# Autodesk Inventor assembly: FrameAssembly
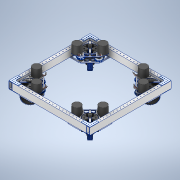
[picture p0: Inventor's stored thumbnail of the model, 180x180]
Saved by Autodesk Inventor 2020 (Build 240168000, 168)
## iProperties
Created: 2019-06-24
Part Number: FrameAssembly
Document SubType Name: Assembly
Designer: Connor
Author: Connor
## Documents named in this file (5)
- C:\Users\Connor\Documents\GrabCAD\2019 Robot\Swerve\TorqyoDriftV2\FrameAssembly.iam
- C:\Users\Connor\Documents\GrabCAD\2019 Robot\Swerve\TorqyoDriftV2\22in2x1Extrusion.ipt
- C:\Users\Connor\Documents\GrabCAD\2019 Robot\Swerve\TorqyoDriftV2\24in2x1Extrusion.ipt
- C:\Users\Connor\Documents\GrabCAD\2019 Robot\Swerve\TorqyoDriftV2\ModuleAssembly.iam
- C:\Users\Connor\Documents\GrabCAD\2019 Robot\Imported Components\VEXPro VersaFrame\General Gussets\90 Degree Gusset.ipt
## Components (16 placed, 4 different names)
1. 22in2x1Extrusion:1 — Mate:1, Flush:1, Flush:2, Flush:6, Flush:11, Flush:13, Insert:2, Insert:9
2. 24in2x1Extrusion:1 — Mate:1, Flush:1, Flush:2, Mate:2, Flush:3, Flush:4, Flush:8, Flush:10, Insert:4, Insert:5, Insert:6, Insert:7, Insert:12, Insert:14, Mate:9, Mate:12, Mate:13
3. 22in2x1Extrusion:2 — Mate:2, Flush:3, Flush:4, Mate:3, Flush:7, Flush:9, Flush:14, Mate:8, Insert:11, Insert:13
4. 24in2x1Extrusion:2 — Flush:6, Mate:3, Flush:7, Flush:12, Flush:15, Insert:1, Insert:3, Insert:8, Insert:10, Mate:10, Mate:11
5. ModuleAssembly:1 [sub-assembly] — Flush:12, Flush:13, Mate:11
6. ModuleAssembly:2 [sub-assembly] — Flush:8, Flush:9, Mate:13
7. ModuleAssembly:3 [sub-assembly] — Flush:14, Flush:15, Mate:10
8. ModuleAssembly:4 [sub-assembly] — Flush:10, Flush:11, Mate:12
9. 90 Degree Gusset:1 — Insert:3, Mate:8
10. 90 Degree Gusset:2 — Insert:8, Insert:9
11. 90 Degree Gusset:3 — Insert:6, Insert:7
12. 90 Degree Gusset:4 — Insert:4, Insert:5
13. 90 Degree Gusset:5 — Insert:10, Insert:11
14. 90 Degree Gusset:6 — Insert:12, Insert:13
15. 90 Degree Gusset:7 — Insert:1, Insert:2
16. 90 Degree Gusset:8 — Insert:14, Mate:9
## Relationships (37: Flush 14, Insert 14, Mate 9)
- Mate:1: 22in2x1Extrusion:1 ↔ 24in2x1Extrusion:1
- Flush:1: 22in2x1Extrusion:1 ↔ 24in2x1Extrusion:1
- Flush:2: 22in2x1Extrusion:1 ↔ 24in2x1Extrusion:1
- Mate:2: 24in2x1Extrusion:1 ↔ 22in2x1Extrusion:2
- Flush:3: 24in2x1Extrusion:1 ↔ 22in2x1Extrusion:2
- Flush:4: 24in2x1Extrusion:1 ↔ 22in2x1Extrusion:2
- Flush:6: 22in2x1Extrusion:1 ↔ 24in2x1Extrusion:2
- Mate:3: 22in2x1Extrusion:2 ↔ 24in2x1Extrusion:2
- Flush:7: 22in2x1Extrusion:2 ↔ 24in2x1Extrusion:2
- Flush:8: 24in2x1Extrusion:1 ↔ ModuleAssembly:2
- Flush:9: 22in2x1Extrusion:2 ↔ ModuleAssembly:2
- Flush:10: 24in2x1Extrusion:1 ↔ ModuleAssembly:4
- Flush:11: 22in2x1Extrusion:1 ↔ ModuleAssembly:4
- Flush:12: 24in2x1Extrusion:2 ↔ ModuleAssembly:1
- Flush:13: 22in2x1Extrusion:1 ↔ ModuleAssembly:1
- Flush:14: 22in2x1Extrusion:2 ↔ ModuleAssembly:3
- Flush:15: 24in2x1Extrusion:2 ↔ ModuleAssembly:3
- Insert:1: 24in2x1Extrusion:2 ↔ 90 Degree Gusset:7
- Insert:2: 22in2x1Extrusion:1 ↔ 90 Degree Gusset:7
- Insert:3: 24in2x1Extrusion:2 ↔ 90 Degree Gusset:1
- Mate:8: 22in2x1Extrusion:2 ↔ 90 Degree Gusset:1
- Insert:4: 24in2x1Extrusion:1 ↔ 90 Degree Gusset:4
- Insert:5: 24in2x1Extrusion:1 ↔ 90 Degree Gusset:4
- Insert:6: 24in2x1Extrusion:1 ↔ 90 Degree Gusset:3
- Insert:7: 24in2x1Extrusion:1 ↔ 90 Degree Gusset:3
- Insert:8: 24in2x1Extrusion:2 ↔ 90 Degree Gusset:2
- Insert:9: 22in2x1Extrusion:1 ↔ 90 Degree Gusset:2
- Insert:10: 24in2x1Extrusion:2 ↔ 90 Degree Gusset:5
- Insert:11: 22in2x1Extrusion:2 ↔ 90 Degree Gusset:5
- Insert:12: 24in2x1Extrusion:1 ↔ 90 Degree Gusset:6
- Insert:13: 22in2x1Extrusion:2 ↔ 90 Degree Gusset:6
- Insert:14: 24in2x1Extrusion:1 ↔ 90 Degree Gusset:8
- Mate:9: 24in2x1Extrusion:1 ↔ 90 Degree Gusset:8
- Mate:10: 24in2x1Extrusion:2 ↔ ModuleAssembly:3
- Mate:11: 24in2x1Extrusion:2 ↔ ModuleAssembly:1
- Mate:12: 24in2x1Extrusion:1 ↔ ModuleAssembly:4
- Mate:13: 24in2x1Extrusion:1 ↔ ModuleAssembly:2
